# Autodesk Inventor assembly: elevation_assembly
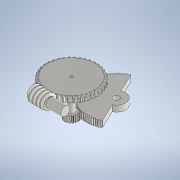
[picture p0: Inventor's stored thumbnail of the model, 180x180]
Saved by Autodesk Inventor 2020 (Build 240168000, 168)
## iProperties
Created: 2020-05-17
Part Number: elevation_assembly
Document SubType Name: Assembly
Designer: Hesekiel
Author: Hesekiel
## Documents named in this file (4)
- C:\Users\Hesekiel\Documents\Inventor\Uchwyt Aktywny Teleskopu\elevation_assembly.iam
- C:\Users\Hesekiel\Documents\Inventor\Uchwyt Aktywny Teleskopu\worm_gear.iam
- C:\Users\Hesekiel\Documents\Inventor\Uchwyt Aktywny Teleskopu\rack_and_pinion.iam
- C:\Users\Hesekiel\Documents\Inventor\Uchwyt Aktywny Teleskopu\wał_elewacji.ipt
## Components (3 placed, 3 different names)
1. worm_gear:1 [sub-assembly] — Rigid:1
2. rack_and_pinion:1 [sub-assembly] — Rigid:2
3. wał_elewacji:1 — Rigid:1, Rigid:2
## Relationships (2: WeldJoint 2)
- Rigid:1 [WeldJoint]: worm_gear:1 ↔ wał_elewacji:1
- Rigid:2 [WeldJoint]: rack_and_pinion:1 ↔ wał_elewacji:1
